# Autodesk Inventor assembly: PWTR-0023
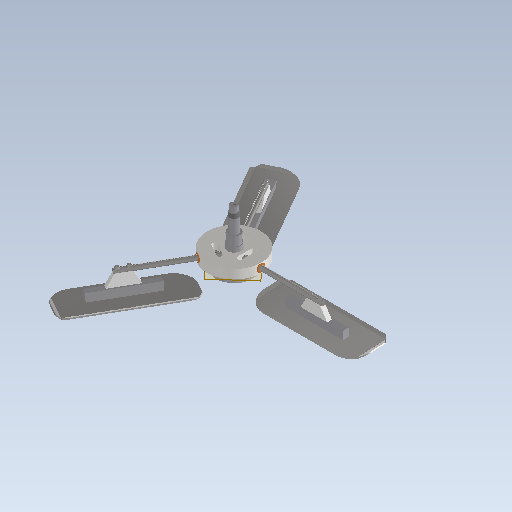
[picture p0: Inventor's stored thumbnail of the model, 512x512]
Saved by Autodesk Inventor 2021.1 (Build 251245010, 245A)
## iProperties
Created: 2019-05-30
Part Number: PWTR-0023
Document SubType Name: Assembly
Designer: alid
Description: Trowel Sub Assembly
Vendor: Design Specific
Author: alid
Revision Number: A
## Documents named in this file (10)
- C:\Users\peter\source\repos\InventorDA-FLC\Dataset\FY2021 Power Trowel\PWTR-0023.iam
- C:\Users\peter\source\repos\InventorDA-FLC\Dataset\FY2021 Power Trowel\PWTR-0032.ipt
- C:\Users\peter\source\repos\InventorDA-FLC\Dataset\FY2021 Power Trowel\PWTR-0035.ipt
- C:\Users\peter\source\repos\InventorDA-FLC\Dataset\FY2021 Power Trowel\PWTR-0026.ipt
- C:\Users\peter\source\repos\InventorDA-FLC\Dataset\FY2021 Power Trowel\PWTR-0037.ipt
- C:\Users\peter\source\repos\InventorDA-FLC\Dataset\FY2021 Power Trowel\PWTR-0038.ipt
- C:\Users\peter\source\repos\InventorDA-FLC\Dataset\FY2021 Power Trowel\PWTR-0044.iam
- C:\Users\peter\source\repos\InventorDA-FLC\Dataset\FY2021 Power Trowel\PWTR-0049.ipt
- C:\Users\peter\source\repos\InventorDA-FLC\Dataset\FY2021 Power Trowel\PWTR-0153.ipt
- C:\Users\peter\source\repos\InventorDA-FLC\Dataset\FY2021 Power Trowel\PWTR-0154.ipt
## Components (16 placed, 9 different names)
1. TROWEL SPIDER — Mate:21, Mate:47, Insert:26
2. LOWER UNIVERSAL — Angle:1, Mate:71
3. PWTR-0037:1 — Angle:1, Mate:70
4. PWTR-0038:1
5. DIN 7984 M5 x 20:5
6. DIN 7984 M5 x 20:6
7. DIN 7984 M5 x 20:7
8. DIN 7984 M5 x 20:8
9. DIN 7984 M6 x 16:1
10. PWTR-0049:1 — Mate:70, Mate:71
11. PWTR-0044:1 [sub-assembly] — Mate:21, Mate:47
12. PWTR-0026:2 — Insert:26
13. PWTR-0044:2 [sub-assembly]
14. PWTR-0026:3
15. PWTR-0044:3 [sub-assembly]
16. PWTR-0026:4
## Component patterns: Trowel Pattern (3 elements)
## Relationships (20: Mate 12, Insert 6, Tangent 1, Angle 1)
- [Mate]: TROWEL SPIDER ↔ LOWER UNIVERSAL
- [Mate]: TROWEL SPIDER ↔ LOWER UNIVERSAL
- [Insert]: TROWEL SPIDER ↔ DIN 7984 M5 x 20:5
- [Insert]: TROWEL SPIDER ↔ DIN 7984 M5 x 20:6
- [Insert]: TROWEL SPIDER ↔ DIN 7984 M5 x 20:7
- [Insert]: TROWEL SPIDER ↔ DIN 7984 M5 x 20:8
- [Mate]: TROWEL SPIDER ↔ LOWER UNIVERSAL
- Mate:21 (0.5 mm): TROWEL SPIDER ↔ PWTR-0044:1
- [Mate]: TROWEL SPIDER ↔ PWTR-0037:1
- [Mate]: PWTR-0037:1 ↔ PWTR-0038:1
- [Mate]: PWTR-0037:1 ↔ PWTR-0038:1
- [Insert]: PWTR-0038:1 ↔ DIN 7984 M6 x 16:1
- [Tangent]: PWTR-0038:1 ↔ PWTR-0044:1
- Mate:47: TROWEL SPIDER ↔ PWTR-0044:1
- [Mate] (20.701 mm): TROWEL SPIDER ↔ PWTR-0038:1
- [Mate]: PWTR-0037:1 ↔ PWTR-0038:1
- Insert:26: TROWEL SPIDER ↔ PWTR-0026:2
- Angle:1 (90 deg): LOWER UNIVERSAL ↔ PWTR-0037:1
- Mate:70: PWTR-0037:1 ↔ PWTR-0049:1
- Mate:71: LOWER UNIVERSAL ↔ PWTR-0049:1
## Named parameters: d0_d1 = 0 mm, d1_d3 = 0 mm, d2_d12 = 0 mm, d70_d82 = 0.5 mm
